# Autodesk Inventor assembly: ENSAMBLE BOMBA
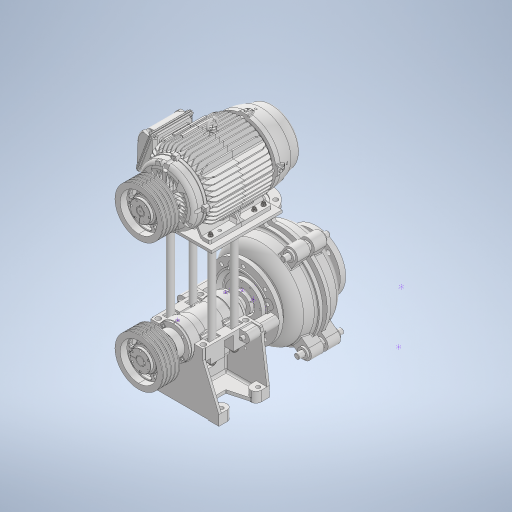
[picture p0: Inventor's stored thumbnail of the model, 512x512]
Saved by Autodesk Inventor 2024.1 (Build 281209000, 209)
## iProperties
Created: 2025-06-24
Part Number: ENSAMBLE BOMBA
Document SubType Name: Assembly
Designer: User
Author: User
## Documents named in this file (12)
- C:\Users\User\OneDrive\Documents\POLEAS\ENSAMBLE BOMBA.iam
- C:\Users\User\OneDrive\Documents\POLEAS\6209K324_Quick-Disconnect Bushing-Bore V-Belt Pulley.iam
- C:\Users\User\OneDrive\Documents\POLEAS\phf_sk-32mm.ipt
- C:\Users\User\OneDrive\Documents\POLEAS\MOTOR ELECTRICO WEG 75 HP\07568453.iam
- C:\Users\User\OneDrive\Documents\POLEAS\WARMAN 4X3 SOPORTE\WARMAN 4_3.iam
- C:\Users\User\OneDrive\Documents\POLEAS\phf_sk-42mm.ipt
- C:\Users\User\OneDrive\Documents\POLEAS\WARMAN 4X3 SOPORTE\PLACA BASE.ipt
- C:\Users\User\OneDrive\Documents\POLEAS\WARMAN 4X3 SOPORTE\BARRA SOPORTE.ipt
- C:\Users\User\OneDrive\Documents\Inventor\Content Center Files\R2024\en-US\DIN 6923\DIN 6923 - M20 x 2,5.ipt
- C:\Users\User\OneDrive\Documents\Inventor\Content Center Files\R2024\en-US\AS 1427(00)\AS 1427 - M10 x 45(4).ipt
- C:\Users\User\OneDrive\Documents\Inventor\Content Center Files\R2024\en-US\DIN 6331\DIN 6331 - M 30.ipt
- C:\Users\User\OneDrive\Documents\Inventor\Content Center Files\R2024\en-US\DIN 6923\DIN 6923 - M10 x 1,25.ipt
## Components (31 placed, 11 different names)
1. 6209K324_Quick-Disconnect Bushing-Bore V-Belt Pulley:1 [sub-assembly] — Flush:1, Flush:2, Flush:3, Mate:1, Mate:2, Flush:10
2. phf_sk-32mm:1 — Mate:1, Mate:2, Flush:7, Flush:11
3. 07568453:1 [sub-assembly] — Flush:4, Flush:5, Flush:6, Flush:7, Mate:3, Flush:9, Mate:7, Flush:13, Mate:12, Mate:14, Mate:20, Mate:22, Mate:24, Mate:26
4. WARMAN 4_3:1 [sub-assembly] — Mate:3, Flush:8, Flush:9, Mate:4, Mate:5, Angle:1, Angle:2, Flush:12, Mate:8, Insert:1, Insert:2, Insert:3, Insert:4
5. phf_sk-42mm:1 — Mate:5, Angle:1, Mate:6, Flush:11
6. 6209K324_Quick-Disconnect Bushing-Bore V-Belt Pulley:2 [sub-assembly] — Mate:4, Flush:10, Mate:6
7. PLACA BASE:1 — Mate:7, Angle:2, Flush:12, Flush:13, Flush:14, Mate:9, Mate:10, Mate:11, Mate:13, Mate:15, Mate:21, Mate:23, Mate:25, Mate:27, Insert:5, Insert:6, Insert:7, Insert:8
8. BARRA SOPORTE:1 — Mate:9, Flush:15
9. BARRA SOPORTE:2 — Mate:10, Flush:16, Flush:17
10. BARRA SOPORTE:3 — Mate:8, Flush:14, Flush:15, Flush:16
11. BARRA SOPORTE:4 — Mate:11, Flush:17
12. DIN 6923 M20:1 — Insert:1
13. DIN 6923 M20:2 — Insert:2
14. DIN 6923 M20:3 — Insert:3
15. DIN 6923 M20:4 — Insert:4
16. AS 1427 - Metric M10 x 45:1 — Mate:12, Mate:13
17. AS 1427 - Metric M10 x 45:2 — Mate:14, Mate:15, Mate:29
18. AS 1427 - Metric M10 x 45:5 — Mate:20, Mate:21
19. AS 1427 - Metric M10 x 45:6 — Mate:22, Mate:23
20. AS 1427 - Metric M10 x 45:7 — Mate:24, Mate:25, Mate:28
21. AS 1427 - Metric M10 x 45:8 — Mate:26, Mate:27, Mate:30
22. DIN 6331 M 30:1 — Insert:5
23. DIN 6331 M 30:2 — Insert:6
24. DIN 6331 M 30:3 — Insert:7
25. DIN 6331 M 30:4 — Insert:8
26. DIN 6923 M10 x 1,25:1 — Mate:28
27. DIN 6923 M10 x 1,25:2 — Mate:29
28. DIN 6923 M10 x 1,25:3 — Mate:30
29. DIN 6923 M10 x 1,25:4
30. DIN 6923 M10 x 1,25:5
31. DIN 6923 M10 x 1,25:6
## Relationships (53: Mate 26, Flush 17, Insert 8, Angle 2)
- Flush:1: 6209K324_Quick-Disconnect Bushing-Bore V-Belt Pulley:1
- Flush:2: 6209K324_Quick-Disconnect Bushing-Bore V-Belt Pulley:1
- Flush:3 (-52 mm): 6209K324_Quick-Disconnect Bushing-Bore V-Belt Pulley:1
- Mate:1: 6209K324_Quick-Disconnect Bushing-Bore V-Belt Pulley:1 ↔ phf_sk-32mm:1
- Mate:2: 6209K324_Quick-Disconnect Bushing-Bore V-Belt Pulley:1 ↔ phf_sk-32mm:1
- Flush:4: 07568453:1
- Flush:5: 07568453:1
- Flush:6 (-200 mm): 07568453:1
- Flush:7: phf_sk-32mm:1 ↔ 07568453:1
- Mate:3 (200 mm): 07568453:1 ↔ WARMAN 4_3:1
- Flush:8: WARMAN 4_3:1
- Flush:9: 07568453:1 ↔ WARMAN 4_3:1
- Mate:4: WARMAN 4_3:1 ↔ 6209K324_Quick-Disconnect Bushing-Bore V-Belt Pulley:2
- Flush:10: 6209K324_Quick-Disconnect Bushing-Bore V-Belt Pulley:1 ↔ 6209K324_Quick-Disconnect Bushing-Bore V-Belt Pulley:2
- Mate:5: WARMAN 4_3:1 ↔ phf_sk-42mm:1
- Angle:1 (0 deg): WARMAN 4_3:1 ↔ phf_sk-42mm:1
- Mate:6: phf_sk-42mm:1 ↔ 6209K324_Quick-Disconnect Bushing-Bore V-Belt Pulley:2
- Flush:11: phf_sk-32mm:1 ↔ phf_sk-42mm:1
- Mate:7: 07568453:1 ↔ PLACA BASE:1
- Angle:2 (0 deg): WARMAN 4_3:1 ↔ PLACA BASE:1
- Flush:12 (-48.936 mm): WARMAN 4_3:1 ↔ PLACA BASE:1
- Flush:13 (-20 mm): 07568453:1 ↔ PLACA BASE:1
- Mate:8: WARMAN 4_3:1 ↔ BARRA SOPORTE:3
- Flush:14: PLACA BASE:1 ↔ BARRA SOPORTE:3
- Mate:9: PLACA BASE:1 ↔ BARRA SOPORTE:1
- Flush:15: BARRA SOPORTE:1 ↔ BARRA SOPORTE:3
- Mate:10: PLACA BASE:1 ↔ BARRA SOPORTE:2
- Flush:16: BARRA SOPORTE:2 ↔ BARRA SOPORTE:3
- Mate:11: PLACA BASE:1 ↔ BARRA SOPORTE:4
- Flush:17: BARRA SOPORTE:2 ↔ BARRA SOPORTE:4
- Insert:1: WARMAN 4_3:1 ↔ DIN 6923 M20:1
- Insert:2: WARMAN 4_3:1 ↔ DIN 6923 M20:2
- Insert:3: WARMAN 4_3:1 ↔ DIN 6923 M20:3
- Insert:4: WARMAN 4_3:1 ↔ DIN 6923 M20:4
- Mate:12: 07568453:1 ↔ AS 1427 - Metric M10 x 45:1
- Mate:13: PLACA BASE:1 ↔ AS 1427 - Metric M10 x 45:1
- Mate:14: 07568453:1 ↔ AS 1427 - Metric M10 x 45:2
- Mate:15: PLACA BASE:1 ↔ AS 1427 - Metric M10 x 45:2
- Mate:20: 07568453:1 ↔ AS 1427 - Metric M10 x 45:5
- Mate:21: PLACA BASE:1 ↔ AS 1427 - Metric M10 x 45:5
- Mate:22: 07568453:1 ↔ AS 1427 - Metric M10 x 45:6
- Mate:23: PLACA BASE:1 ↔ AS 1427 - Metric M10 x 45:6
- Mate:24: 07568453:1 ↔ AS 1427 - Metric M10 x 45:7
- Mate:25: PLACA BASE:1 ↔ AS 1427 - Metric M10 x 45:7
- Mate:26: 07568453:1 ↔ AS 1427 - Metric M10 x 45:8
- Mate:27: PLACA BASE:1 ↔ AS 1427 - Metric M10 x 45:8
- Insert:5: PLACA BASE:1 ↔ DIN 6331 M 30:1
- Insert:6: PLACA BASE:1 ↔ DIN 6331 M 30:2
- Insert:7: PLACA BASE:1 ↔ DIN 6331 M 30:3
- Insert:8: PLACA BASE:1 ↔ DIN 6331 M 30:4
- Mate:28: AS 1427 - Metric M10 x 45:7 ↔ DIN 6923 M10 x 1,25:1
- Mate:29: AS 1427 - Metric M10 x 45:2 ↔ DIN 6923 M10 x 1,25:2
- Mate:30: AS 1427 - Metric M10 x 45:8 ↔ DIN 6923 M10 x 1,25:3
